# Autodesk Inventor assembly: New Final Leg Assembly
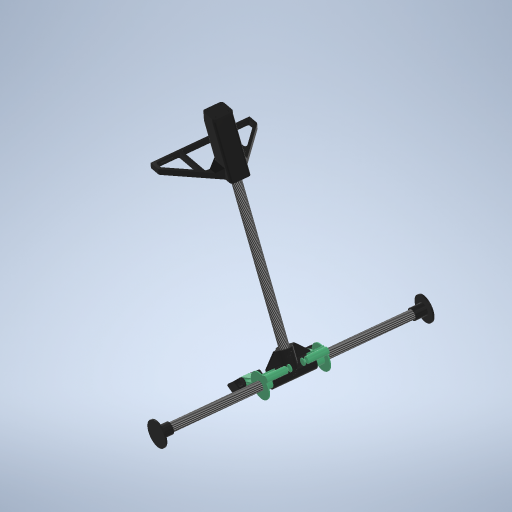
[picture p0: Inventor's stored thumbnail of the model, 512x512]
Saved by Autodesk Inventor 2023 (Build 270158000, 158)
## iProperties
Created: 2023-01-21
Part Number: New Final Leg Assembly
Document SubType Name: Assembly
Designer: chase
Author: chase
## Documents named in this file (9)
- D:\Documents\GitHub\WU-Team20-AutonomousDrone\CAD\ASSEMBLY\SubAssembly - Leg SingleSide.iam
- D:\Documents\GitHub\WU-Team20-AutonomousDrone\CAD\Legs\UpperLandingLegMount - Shortened+WebBrace+Lightened.ipt
- D:\Documents\GitHub\WU-Team20-AutonomousDrone\CAD\Raw Models\CarbonTube - 16ODx373mm.ipt
- D:\Documents\GitHub\WU-Team20-AutonomousDrone\CAD\Legs\LegTeeJoint - 16x16mmHoles.ipt
- D:\Documents\GitHub\WU-Team20-AutonomousDrone\CAD\Raw Models\CarbonTube - 16ODx457,2mm.ipt
- D:\Documents\GitHub\WU-Team20-AutonomousDrone\CAD\Legs\ChargingArm - FlatPlate.ipt
- D:\Documents\GitHub\WU-Team20-AutonomousDrone\CAD\Legs\Leg EndCap - ForPoolNoodle.ipt
- D:\Documents\GitHub\WU-Team20-AutonomousDrone\CAD\Legs\ChargingArm - FlatPlateBracket.ipt
- D:\Documents\GitHub\WU-Team20-AutonomousDrone\CAD\Legs\ChargingArm - FlatPlate_MIR.ipt
## Components (12 placed, 8 different names)
1. UpperLandingLegMount - Shortened+WebBrace+Lightened:1 — Insert:4, Angle:1
2. CarbonTube - 16ODx373mm:1 — Insert:2, Insert:4
3. LegTeeJoint - 16x16mmHoles:1 — Insert:2, Insert:3, Rotational:1, Rotational:3, Angle:1
4. CarbonTube - 16ODx457,2mm:1 — Insert:3, Rigid:1, Rigid:2
5. ChargingArm - FlatPlate:1 — Rotational:1, Rotational:2, Flush:1, Rotational:4
6. Leg EndCap - ForPoolNoodle:1 — Rigid:1
7. ChargingArm - FlatPlateBracket:1 — Rotational:2, Flush:2, Flush:3, Flush:4
8. Leg EndCap - ForPoolNoodle:2 — Rigid:2
9. ChargingArm - FlatPlate_MIR:1 — Rotational:3, Flush:1, Rotational:5, Rotational:6
10. ChargingArm - FlatPlateBracket:2 — Rotational:6, Flush:3
11. ChargingArm - FlatPlateBracket:3 — Rotational:4, Flush:2
12. ChargingArm - FlatPlateBracket:4 — Rotational:5, Flush:4
## Relationships (16: RevoluteJoint 6, Flush 4, Insert 3, WeldJoint 2, Angle 1)
- Insert:2: CarbonTube - 16ODx373mm:1 ↔ LegTeeJoint - 16x16mmHoles:1
- Insert:3 (-191.1 mm): LegTeeJoint - 16x16mmHoles:1 ↔ CarbonTube - 16ODx457,2mm:1
- Insert:4: UpperLandingLegMount - Shortened+WebBrace+Lightened:1 ↔ CarbonTube - 16ODx373mm:1
- Rotational:1 [RevoluteJoint]: LegTeeJoint - 16x16mmHoles:1 ↔ ChargingArm - FlatPlate:1
- Rigid:1 [WeldJoint]: CarbonTube - 16ODx457,2mm:1 ↔ Leg EndCap - ForPoolNoodle:1
- Rotational:2 [RevoluteJoint]: ChargingArm - FlatPlate:1 ↔ ChargingArm - FlatPlateBracket:1
- Rigid:2 [WeldJoint]: CarbonTube - 16ODx457,2mm:1 ↔ Leg EndCap - ForPoolNoodle:2
- Rotational:3 [RevoluteJoint]: LegTeeJoint - 16x16mmHoles:1 ↔ ChargingArm - FlatPlate_MIR:1
- Flush:1: ChargingArm - FlatPlate:1 ↔ ChargingArm - FlatPlate_MIR:1
- Rotational:4 [RevoluteJoint]: ChargingArm - FlatPlate:1 ↔ ChargingArm - FlatPlateBracket:3
- Rotational:5 [RevoluteJoint]: ChargingArm - FlatPlate_MIR:1 ↔ ChargingArm - FlatPlateBracket:4
- Rotational:6 [RevoluteJoint]: ChargingArm - FlatPlate_MIR:1 ↔ ChargingArm - FlatPlateBracket:2
- Flush:2: ChargingArm - FlatPlateBracket:1 ↔ ChargingArm - FlatPlateBracket:3
- Flush:3: ChargingArm - FlatPlateBracket:1 ↔ ChargingArm - FlatPlateBracket:2
- Flush:4: ChargingArm - FlatPlateBracket:1 ↔ ChargingArm - FlatPlateBracket:4
- Angle:1 (0 deg): UpperLandingLegMount - Shortened+WebBrace+Lightened:1 ↔ LegTeeJoint - 16x16mmHoles:1
